# Autodesk Inventor assembly: frame printer
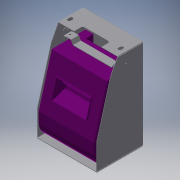
[picture p0: Inventor's stored thumbnail of the model, 180x180]
Saved by Autodesk Inventor 2016 (Build 200138000, 138)
## iProperties
Created: 2018-11-14
Part Number: frame printer
Document SubType Name: Assembly
Designer: hovm
Author: hovm
## Documents named in this file (5)
- C:\Users\hovm\Desktop\DaoCM's project\frame printer.iam
- C:\Users\hovm\Desktop\DaoCM's project\Part105.ipt
- C:\Users\hovm\Desktop\DaoCM's project\printer2.ipt
- C:\Users\hovm\Desktop\DaoCM's project\Part106.ipt
- C:\Users\hovm\Desktop\DaoCM's project\Part107.ipt
## Components (5 placed, 4 different names)
1. Part105:3 — Mate:1, Mate:2, Mate:3, Mate:4, Mate:6
2. printer2:1 — Mate:1, Mate:2, Mate:3, Flush:1
3. Part106:1 — Flush:1, Flush:2, Mate:5, Mate:7, Flush:3
4. Part107:1 — Mate:4, Flush:2, Mate:5
5. Part107:2 — Mate:6, Mate:7, Flush:3
## Relationships (10: Mate 7, Flush 3)
- Mate:1 (1 mm): Part105:3 ↔ printer2:1
- Mate:2 (3 mm): Part105:3 ↔ printer2:1
- Mate:3: Part105:3 ↔ printer2:1
- Flush:1 (1 mm): printer2:1 ↔ Part106:1
- Mate:4: Part105:3 ↔ Part107:1
- Flush:2: Part106:1 ↔ Part107:1
- Mate:5: Part106:1 ↔ Part107:1
- Mate:6: Part105:3 ↔ Part107:2
- Mate:7: Part106:1 ↔ Part107:2
- Flush:3: Part106:1 ↔ Part107:2
